# Autodesk Inventor assembly: ASSY,ROBOT,2026
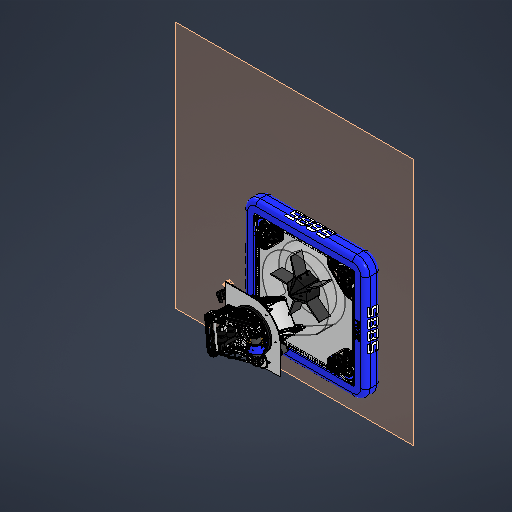
[picture p0: Inventor's stored thumbnail of the model, 512x512]
Saved by Autodesk Inventor 2026 (Build 300175000, 175)
## iProperties
Created: 2026-01-24
Part Number: ASSY,ROBOT,2026
Document SubType Name: Assembly
Designer: Jthib
Mass: 39497.7 g
Surface Area: 76984.5 cm^2
Volume: 36761.1 cm^3
Density: 1.07444 g/cm^3
Author: Jthib
## Documents named in this file (6)
- C:\Users\littl\OneDrive\Documents\GitHub\2026-Robot-Mechanical\ASSY,ROBOT,2026.iam
- C:\Users\littl\OneDrive\Documents\GitHub\2026-Robot-Mechanical\Chassis\CHASSIS.iam
- C:\Users\littl\OneDrive\Documents\GitHub\2026-Robot-Mechanical\Chassis\Bumpers.ipt
- C:\Users\littl\OneDrive\Documents\GitHub\2026-Robot-Mechanical\Spindexer\#Spindexer.iam
- C:\Users\littl\OneDrive\Documents\GitHub\2026-Robot-Mechanical\Shooter\Shooter - Front Motors\#SHOOTER.FRONT_MOTORS.iam
- C:\Users\littl\OneDrive\Documents\GitHub\2026-Robot-Mechanical\Shooter\Turret\#Turret.iam
## Components (5 placed, 5 different names)
1. CHASSIS:1 [sub-assembly] — Flush:1, Flush:2, Flush:3, Flush:4, Mate:1, Mate:2, Mate:9, Mate:10, Mate:11, Tangent:1, Mate:13
2. Bumpers:1 — Flush:4, Mate:1, Mate:2
3. #Spindexer:1 [sub-assembly] — Mate:11, Mate:12, Tangent:1, Mate:13, Mate:14, Mate:16
4. #SHOOTER.FRONT_MOTORS:1 [sub-assembly] — Mate:9, Mate:10, Mate:12, Mate:15, Mate:17
5. #Turret:1 [sub-assembly] — Mate:14, Mate:15, Mate:16, Mate:17
## Relationships (16: Mate 11, Flush 4, Tangent 1)
- Flush:1 (-349.25 mm): CHASSIS:1
- Flush:2 (349.25 mm): CHASSIS:1
- Flush:3: CHASSIS:1
- Flush:4 (-12.7 mm): CHASSIS:1 ↔ Bumpers:1
- Mate:1: CHASSIS:1 ↔ Bumpers:1
- Mate:2: CHASSIS:1 ↔ Bumpers:1
- Mate:9 (-190.5 mm): CHASSIS:1 ↔ #SHOOTER.FRONT_MOTORS:1
- Mate:10 (-190.5 mm): CHASSIS:1 ↔ #SHOOTER.FRONT_MOTORS:1
- Mate:11: CHASSIS:1 ↔ #Spindexer:1
- Mate:12 (79.375 mm): #Spindexer:1 ↔ #SHOOTER.FRONT_MOTORS:1
- Tangent:1: CHASSIS:1 ↔ #Spindexer:1
- Mate:13 (-304.8 mm): CHASSIS:1 ↔ #Spindexer:1
- Mate:14: #Spindexer:1 ↔ #Turret:1
- Mate:15: #SHOOTER.FRONT_MOTORS:1 ↔ #Turret:1
- Mate:16: #Spindexer:1 ↔ #Turret:1
- Mate:17: #SHOOTER.FRONT_MOTORS:1 ↔ #Turret:1
